# Autodesk Inventor assembly: 40 направляшка
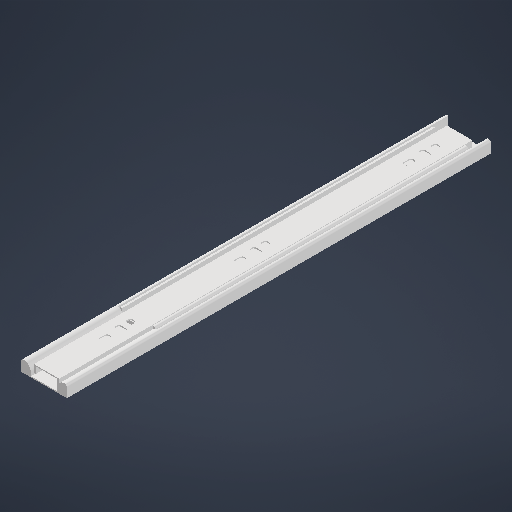
[picture p0: Inventor's stored thumbnail of the model, 512x512]
Saved by Autodesk Inventor 2025 (Build 290162000, 162)
## iProperties
Created: 2024-12-03
Part Number: 40 направляшка
Document SubType Name: Assembly
Designer: Phantom
Author: Phantom
## Documents named in this file (4)
- C:\Users\Phantom\Desktop\Phantom16950\40 направляшка.iam
- C:\Users\Phantom\Desktop\Phantom16950\3 часть направляшки.ipt
- C:\Users\Phantom\Desktop\Phantom16950\2 часть направляшки.ipt
- C:\Users\Phantom\Desktop\Phantom16950\1 часть направляшки.ipt
## Components (3 placed, 3 different names)
1. 3 часть направляшки:1 — Совмещение:3, Совмещение:4
2. 2 часть направляшки:1 — Совмещение:1, Совмещение:2, Совмещение:3, Совмещение:4
3. 1 часть направляшки:1 — Совмещение:1, Совмещение:2
## Relationships (4: Mate 4)
- Совмещение:1 [Mate]: 2 часть направляшки:1 ↔ 1 часть направляшки:1
- Совмещение:2 [Mate]: 2 часть направляшки:1 ↔ 1 часть направляшки:1
- Совмещение:3 [Mate]: 3 часть направляшки:1 ↔ 2 часть направляшки:1
- Совмещение:4 [Mate]: 3 часть направляшки:1 ↔ 2 часть направляшки:1
